# Autodesk Inventor assembly: brazo conexion
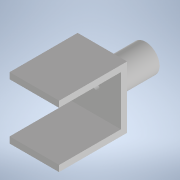
[picture p0: Inventor's stored thumbnail of the model, 180x180]
Saved by Autodesk Inventor 2020.3 (Build 243373000, 373)
## iProperties
Created: 2021-02-09
Part Number: brazo conexion
Document SubType Name: Assembly
Designer: Yu Jinyu
Author: Yu Jinyu
## Documents named in this file (3)
- C:\Users\Yu Jinyu\OneDrive\Escritorio\Yaw Roll Nuevo\brazo conexion.iam
- C:\Users\Yu Jinyu\OneDrive\Escritorio\Yaw Roll Nuevo\brazo.ipt
- C:\Users\Yu Jinyu\OneDrive\Escritorio\Yaw Roll Nuevo\tubo.ipt
## Components (2 placed, 2 different names)
1. brazo:1 — Insert:1
2. tubo:1 — Insert:1
## Relationships (1: Insert 1)
- Insert:1: brazo:1 ↔ tubo:1
